# Autodesk Inventor assembly: My First Assembly
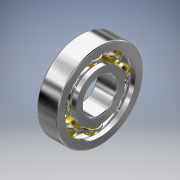
[picture p0: Inventor's stored thumbnail of the model, 180x180]
Saved by Autodesk Inventor 2018 (Build 220112000, 112)
## iProperties
Created: 2019-07-01
Part Number: My First Assembly
Document SubType Name: Assembly
Designer: HP
Author: HP
## Documents named in this file (5)
- C:\Users\Sameer\Desktop\Saad\SMA\Ball Bearing\My First Assembly.iam
- C:\Users\Sameer\Desktop\Saad\SMA\Ball Bearing\Outer Rings.ipt
- C:\Users\Sameer\Desktop\Saad\SMA\Ball Bearing\Inner Ring.ipt
- C:\Users\Sameer\Desktop\Saad\SMA\Ball Bearing\Ball.ipt
- C:\Users\Sameer\Desktop\Saad\SMA\Ball Bearing\Cage.ipt
## Components (11 placed, 4 different names)
1. Outer Rings:1 — Mate:1, Flush:1
2. Inner Ring:1 — Mate:1, Flush:1, Tangent:1, Mate:3, Mate:5
3. Cage:1 — Mate:4, Mate:5, Mate:6
4. Ball:1 — Mate:2, Tangent:1, Mate:3, Mate:6
5. Ball:2
6. Ball:3
7. Ball:4
8. Ball:5
9. Ball:6
10. Ball:7
11. Ball:8
## Component patterns: (8 elements, first: Ball:1)
## Relationships (8: Mate 6, Flush 1, Tangent 1)
- Mate:1: Outer Rings:1 ↔ Inner Ring:1
- Flush:1: Outer Rings:1 ↔ Inner Ring:1
- Mate:2: Ball:1
- Tangent:1: Inner Ring:1 ↔ Ball:1
- Mate:3: Inner Ring:1 ↔ Ball:1
- Mate:4: Cage:1
- Mate:5: Inner Ring:1 ↔ Cage:1
- Mate:6: Cage:1 ↔ Ball:1
